# Autodesk Inventor assembly: extruder
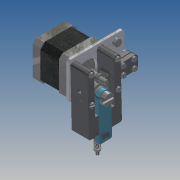
[picture p0: Inventor's stored thumbnail of the model, 180x180]
Saved by Autodesk Inventor 2015 SP1 (Build 190203100, 203)
## iProperties
Created: 2015-01-28
Part Number: extruder
Document SubType Name: Assembly
Designer: Marc
Author: Marc
## Documents named in this file (21)
- E:\Modellflieger\3D Drucker\Motedis300\Extruder\extruder.iam
- E:\Modellflieger\3D Drucker\Motedis300\Extruder\Kugellager-Schieber-Seite.ipt
- C:\Users\Marc\Documents\Inventor\Content Center Files\R2015\de-DE\DIN 125-1  A\DIN 125 - A 8,4.ipt
- E:\Modellflieger\3D Drucker\Motedis300\Kugellager_8x22x7_608ZZ.ipt
- E:\Modellflieger\3D Drucker\Motedis300\Extruder\Drückbrücke.ipt
- E:\Modellflieger\3D Drucker\Motedis300\Extruder\Nema17_Montageplatte_Extruder.ipt
- E:\Modellflieger\3D Drucker\Motedis300\Extruder\Drückbrücke_U.ipt
- E:\Modellflieger\3D Drucker\Motedis300\Nema17 Schrittmotor\Nema17_Schrittmotor.iam
- E:\Modellflieger\3D Drucker\Motedis300\Extruder\MK8_Drive_gear.ipt
- C:\Users\Marc\Documents\Inventor\Content Center Files\R2015\de-DE\DIN 125-1  A\DIN 125 - A 3,7.ipt
- E:\Modellflieger\3D Drucker\Motedis300\Extruder\Kugellager-Schieber-Druckplatte.ipt
- C:\Users\Marc\Documents\Inventor\Content Center Files\R2015\de-DE\DIN 934\DIN 934 - M3 x 0,5.ipt
- E:\Modellflieger\3D Drucker\Motedis300\Extruder\Kugellager-Schieber-Seite_M8Gewinde.ipt
- E:\Modellflieger\3D Drucker\Motedis300\Extruder\Feder.ipt
- C:\Users\Marc\Documents\Inventor\Content Center Files\R2015\de-DE\DIN 125-1  A\DIN 125 - A 3,2.ipt
- C:\Users\Marc\Documents\Inventor\Content Center Files\R2015\de-DE\DIN 84\DIN 84 - M8 x 20.ipt
- C:\Users\Marc\Documents\Inventor\Content Center Files\R2015\de-DE\DIN 84\DIN 84 - M3 x 28.ipt
- E:\Modellflieger\3D Drucker\Motedis300\Extruder\M3x40_Gewindestück.ipt
- C:\Users\Marc\Documents\Inventor\Content Center Files\R2015\de-DE\DIN 84\DIN 84 - M5 x 8.ipt
- C:\Users\Marc\Documents\Inventor\Content Center Files\R2015\de-DE\DIN 84\DIN 84 - M3 x 12.ipt
- E:\Modellflieger\3D Drucker\Motedis300\Extruder\Drückbrücke_U_Gespiegelt.ipt
## Components (39 placed, 20 different names)
1. Kugellager-Schieber-Seite_M8Gewinde:1 — Fluchtend:1, Passend:15, Einfügen:36, Passend:20
2. DIN 125-1 A A 8,4:1 — Einfügen:2, Einfügen:36
3. Kugellager_8x22x7_608ZZ:1 — Einfügen:2, Einfügen:3
4. DIN 125-1 A A 8,4:2 — Einfügen:3, Einfügen:35
5. Kugellager-Schieber-Seite:2 — Fluchtend:1, Passend:9, Fluchtend:8, Passend:11, Einfügen:30, Einfügen:35
6. Nema17_Montageplatte_Extruder:1 — Passend:6, Passend:7, Passend:8, Einfügen:16, Einfügen:17, Einfügen:39, Einfügen:40, Einfügen:43, Einfügen:44
7. Drückbrücke:3 — Einfügen:12, Passend:9, Einfügen:42
8. Drückbrücke:5 — Einfügen:13, Fluchtend:6, Einfügen:41
9. Drückbrücke_U:1 — Einfügen:12, Einfügen:13, Fluchtend:6, Einfügen:25, Einfügen:26, Passend:12, Passend:13, Passend:14, Passend:15, Passend:16, Passend:26, Passend:28, Passend:30, Passend:32
10. Nema17_Schrittmotor:1 [sub-assembly] — Einfügen:16, Einfügen:17, Einfügen:18
11. MK8_Drive_gear:1 — Einfügen:18
12. DIN 125-1 A A 3,7:4
13. DIN 125-1 A A 3,7:6 — Einfügen:42
14. Drückbrücke:6 — Einfügen:28, Fluchtend:10, Einfügen:33, Einfügen:34
15. Drückbrücke:7 — Einfügen:27, Fluchtend:9, Einfügen:31, Einfügen:32
16. Kugellager-Schieber-Druckplatte:1 — Fluchtend:8, Passend:11, Passend:16, Passend:20, Einfügen:37, Passend:22
17. DIN 934 - ersetzt durch DIN EN 24032/28673/28674 M3:1 — Passend:12, Passend:13, Passend:14
18. Drückbrücke_U_Gespiegelt:1 — Einfügen:25, Einfügen:26, Einfügen:27, Fluchtend:9, Einfügen:28, Fluchtend:10, Einfügen:45, Einfügen:46, Einfügen:47, Einfügen:48
19. M3x40_Gewindestück:1 — Einfügen:37, Passend:21, Einfügen:38, Passend:23
20. Feder:1 — Passend:21, Passend:22
21. DIN 125-1 A A 3,2:1 — Einfügen:38, Passend:24
22. DIN 84 - ersetzt durch DIN EN ISO 1207 M8 x 20:1 — Einfügen:30
23. DIN 84 - ersetzt durch DIN EN ISO 1207 M3 x 28:1 — Einfügen:32
24. DIN 84 - ersetzt durch DIN EN ISO 1207 M3 x 28:2 — Einfügen:34
25. DIN 84 - ersetzt durch DIN EN ISO 1207 M3 x 28:3 — Einfügen:31
26. DIN 84 - ersetzt durch DIN EN ISO 1207 M3 x 28:4 — Einfügen:33
27. DIN 934 - ersetzt durch DIN EN 24032/28673/28674 M3:2 — Passend:23, Passend:24
28. DIN 125-1 A A 3,7:7 — Einfügen:39, Einfügen:41
29. DIN 125-1 A A 3,7:8 — Einfügen:40
30. DIN 84 - ersetzt durch DIN EN ISO 1207 M5 x 8:1 — Einfügen:43
31. DIN 84 - ersetzt durch DIN EN ISO 1207 M5 x 8:2 — Einfügen:44
32. DIN 84 - ersetzt durch DIN EN ISO 1207 M3 x 12:1 — Einfügen:45, Passend:29
33. DIN 84 - ersetzt durch DIN EN ISO 1207 M3 x 12:2 — Einfügen:46, Passend:31
34. DIN 84 - ersetzt durch DIN EN ISO 1207 M3 x 12:3 — Einfügen:47, Passend:25
35. DIN 84 - ersetzt durch DIN EN ISO 1207 M3 x 12:4 — Einfügen:48, Passend:27
36. DIN 934 - ersetzt durch DIN EN 24032/28673/28674 M3:3 — Passend:25, Passend:26
37. DIN 934 - ersetzt durch DIN EN 24032/28673/28674 M3:4 — Passend:27, Passend:28
38. DIN 934 - ersetzt durch DIN EN 24032/28673/28674 M3:5 — Passend:29, Passend:30
39. DIN 934 - ersetzt durch DIN EN 24032/28673/28674 M3:6 — Passend:31, Passend:32
## Relationships (58: Insert 30, Mate 23, Flush 5)
- Einfügen:2 [Insert]: DIN 125-1 A A 8,4:1 ↔ Kugellager_8x22x7_608ZZ:1
- Einfügen:3 [Insert]: Kugellager_8x22x7_608ZZ:1 ↔ DIN 125-1 A A 8,4:2
- Fluchtend:1 [Flush]: Kugellager-Schieber-Seite_M8Gewinde:1 ↔ Kugellager-Schieber-Seite:2
- Einfügen:12 [Insert]: Drückbrücke:3 ↔ Drückbrücke_U:1
- Einfügen:13 [Insert]: Drückbrücke:5 ↔ Drückbrücke_U:1
- Passend:6 [Mate]: Nema17_Montageplatte_Extruder:1
- Passend:7 [Mate]: Nema17_Montageplatte_Extruder:1
- Passend:8 [Mate]: Nema17_Montageplatte_Extruder:1
- Passend:9 [Mate]: Kugellager-Schieber-Seite:2 ↔ Drückbrücke:3
- Einfügen:16 [Insert]: Nema17_Montageplatte_Extruder:1 ↔ Nema17_Schrittmotor:1
- Einfügen:17 [Insert]: Nema17_Montageplatte_Extruder:1 ↔ Nema17_Schrittmotor:1
- Einfügen:18 [Insert] (5 mm): Nema17_Schrittmotor:1 ↔ MK8_Drive_gear:1
- Fluchtend:6 [Flush]: Drückbrücke:5 ↔ Drückbrücke_U:1
- Fluchtend:8 [Flush]: Kugellager-Schieber-Seite:2 ↔ Kugellager-Schieber-Druckplatte:1
- Passend:11 [Mate]: Kugellager-Schieber-Seite:2 ↔ Kugellager-Schieber-Druckplatte:1
- Einfügen:25 [Insert]: Drückbrücke_U:1 ↔ Drückbrücke_U_Gespiegelt:1
- Einfügen:26 [Insert]: Drückbrücke_U:1 ↔ Drückbrücke_U_Gespiegelt:1
- Passend:12 [Mate]: Drückbrücke_U:1 ↔ DIN 934 - ersetzt durch DIN EN 24032/28673/28674 M3:1
- Passend:13 [Mate]: Drückbrücke_U:1 ↔ DIN 934 - ersetzt durch DIN EN 24032/28673/28674 M3:1
- Passend:14 [Mate]: Drückbrücke_U:1 ↔ DIN 934 - ersetzt durch DIN EN 24032/28673/28674 M3:1
- Einfügen:27 [Insert]: Drückbrücke:7 ↔ Drückbrücke_U_Gespiegelt:1
- Fluchtend:9 [Flush]: Drückbrücke:7 ↔ Drückbrücke_U_Gespiegelt:1
- Einfügen:28 [Insert]: Drückbrücke:6 ↔ Drückbrücke_U_Gespiegelt:1
- Fluchtend:10 [Flush]: Drückbrücke:6 ↔ Drückbrücke_U_Gespiegelt:1
- Passend:15 [Mate]: Kugellager-Schieber-Seite_M8Gewinde:1 ↔ Drückbrücke_U:1
- Passend:16 [Mate] (2.5 mm): Drückbrücke_U:1 ↔ Kugellager-Schieber-Druckplatte:1
- Einfügen:30 [Insert]: Kugellager-Schieber-Seite:2 ↔ DIN 84 - ersetzt durch DIN EN ISO 1207 M8 x 20:1
- Einfügen:31 [Insert]: Drückbrücke:7 ↔ DIN 84 - ersetzt durch DIN EN ISO 1207 M3 x 28:3
- Einfügen:32 [Insert]: Drückbrücke:7 ↔ DIN 84 - ersetzt durch DIN EN ISO 1207 M3 x 28:1
- Einfügen:33 [Insert]: Drückbrücke:6 ↔ DIN 84 - ersetzt durch DIN EN ISO 1207 M3 x 28:4
- Einfügen:34 [Insert]: Drückbrücke:6 ↔ DIN 84 - ersetzt durch DIN EN ISO 1207 M3 x 28:2
- Einfügen:35 [Insert]: DIN 125-1 A A 8,4:2 ↔ Kugellager-Schieber-Seite:2
- Einfügen:36 [Insert]: Kugellager-Schieber-Seite_M8Gewinde:1 ↔ DIN 125-1 A A 8,4:1
- Passend:20 [Mate]: Kugellager-Schieber-Seite_M8Gewinde:1 ↔ Kugellager-Schieber-Druckplatte:1
- Einfügen:37 [Insert] (-18.4 mm): Kugellager-Schieber-Druckplatte:1 ↔ M3x40_Gewindestück:1
- Passend:21 [Mate]: M3x40_Gewindestück:1 ↔ Feder:1
- Passend:22 [Mate]: Kugellager-Schieber-Druckplatte:1 ↔ Feder:1
- Einfügen:38 [Insert] (-7 mm): M3x40_Gewindestück:1 ↔ DIN 125-1 A A 3,2:1
- Passend:23 [Mate]: M3x40_Gewindestück:1 ↔ DIN 934 - ersetzt durch DIN EN 24032/28673/28674 M3:2
- Passend:24 [Mate]: DIN 125-1 A A 3,2:1 ↔ DIN 934 - ersetzt durch DIN EN 24032/28673/28674 M3:2
- Einfügen:39 [Insert]: Nema17_Montageplatte_Extruder:1 ↔ DIN 125-1 A A 3,7:7
- Einfügen:40 [Insert]: Nema17_Montageplatte_Extruder:1 ↔ DIN 125-1 A A 3,7:8
- Einfügen:41 [Insert]: Drückbrücke:5 ↔ DIN 125-1 A A 3,7:7
- Einfügen:42 [Insert]: Drückbrücke:3 ↔ DIN 125-1 A A 3,7:6
- Einfügen:43 [Insert]: Nema17_Montageplatte_Extruder:1 ↔ DIN 84 - ersetzt durch DIN EN ISO 1207 M5 x 8:1
- Einfügen:44 [Insert]: Nema17_Montageplatte_Extruder:1 ↔ DIN 84 - ersetzt durch DIN EN ISO 1207 M5 x 8:2
- Einfügen:45 [Insert]: Drückbrücke_U_Gespiegelt:1 ↔ DIN 84 - ersetzt durch DIN EN ISO 1207 M3 x 12:1
- Einfügen:46 [Insert]: Drückbrücke_U_Gespiegelt:1 ↔ DIN 84 - ersetzt durch DIN EN ISO 1207 M3 x 12:2
- Einfügen:47 [Insert]: Drückbrücke_U_Gespiegelt:1 ↔ DIN 84 - ersetzt durch DIN EN ISO 1207 M3 x 12:3
- Einfügen:48 [Insert]: Drückbrücke_U_Gespiegelt:1 ↔ DIN 84 - ersetzt durch DIN EN ISO 1207 M3 x 12:4
- Passend:25 [Mate]: DIN 84 - ersetzt durch DIN EN ISO 1207 M3 x 12:3 ↔ DIN 934 - ersetzt durch DIN EN 24032/28673/28674 M3:3
- Passend:26 [Mate]: Drückbrücke_U:1 ↔ DIN 934 - ersetzt durch DIN EN 24032/28673/28674 M3:3
- Passend:27 [Mate]: DIN 84 - ersetzt durch DIN EN ISO 1207 M3 x 12:4 ↔ DIN 934 - ersetzt durch DIN EN 24032/28673/28674 M3:4
- Passend:28 [Mate]: Drückbrücke_U:1 ↔ DIN 934 - ersetzt durch DIN EN 24032/28673/28674 M3:4
- Passend:29 [Mate]: DIN 84 - ersetzt durch DIN EN ISO 1207 M3 x 12:1 ↔ DIN 934 - ersetzt durch DIN EN 24032/28673/28674 M3:5
- Passend:30 [Mate]: Drückbrücke_U:1 ↔ DIN 934 - ersetzt durch DIN EN 24032/28673/28674 M3:5
- Passend:31 [Mate]: DIN 84 - ersetzt durch DIN EN ISO 1207 M3 x 12:2 ↔ DIN 934 - ersetzt durch DIN EN 24032/28673/28674 M3:6
- Passend:32 [Mate]: Drückbrücke_U:1 ↔ DIN 934 - ersetzt durch DIN EN 24032/28673/28674 M3:6
